# Autodesk Inventor assembly: motor
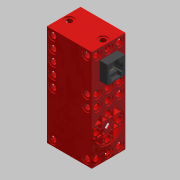
[picture p0: Inventor's stored thumbnail of the model, 180x180]
Saved by Autodesk Inventor 2019.3 (Build 233278000, 278)
## iProperties
Created: 2019-03-27
Part Number: motor
Description: STEP AP214
Document SubType Name: Assembly
Designer: Varga Daniel
Sending System: SolidWorks 2019
Preprocessor: SwSTEP 2.0
Title: motor_.STEP
Revision Number: ANY
## Documents named in this file (10)
- C:\!_Dani\!_cloud\OneDrive\!_munka\Revolution\RevvyDemoKit\Structural parts\Kickstarter videos\Motor\motor.iam
- C:\!_Dani\!_cloud\OneDrive\!_munka\Revolution\RevvyDemoKit\Structural parts\Kickstarter videos\Motor\rj45_vert.ipt
- C:\!_Dani\!_cloud\OneDrive\!_munka\Revolution\RevvyDemoKit\Structural parts\Kickstarter videos\Motor\MOhA.ipt
- C:\!_Dani\!_cloud\OneDrive\!_munka\Revolution\RevvyDemoKit\Structural parts\Kickstarter videos\Motor\MOcA_1.ipt
- C:\!_Dani\!_cloud\OneDrive\!_munka\Revolution\RevvyDemoKit\Structural parts\Kickstarter videos\Motor\MOcA_2.ipt
- C:\!_Dani\!_cloud\OneDrive\!_munka\Revolution\RevvyDemoKit\Structural parts\Kickstarter videos\Motor\ff130-13200.ipt
- C:\!_Dani\!_cloud\OneDrive\!_munka\Revolution\RevvyDemoKit\Structural parts\Kickstarter videos\Motor\Magnet_ring^motor.ipt
- C:\!_Dani\!_cloud\OneDrive\!_munka\Revolution\RevvyDemoKit\Structural parts\Kickstarter videos\Motor\gearbox^motor.ipt
- C:\!_Dani\!_cloud\OneDrive\!_munka\Revolution\RevvyDemoKit\Structural parts\Kickstarter videos\Motor\PCB^motor.ipt
- C:\!_Dani\!_cloud\OneDrive\!_munka\Revolution\RevvyDemoKit\Structural parts\Kickstarter videos\Motor\small_gear.ipt
## Components (10 placed, 10 different names)
1. rj45_vert_1
2. MOhA_2
3. MOhA_3
4. MOcA_1_4
5. MOcA_2_5
6. ff130-13200_6 — Flush:1, Flush:2, Mate:1, Mate:2, Flush:3, Mate:3, Flush:4
7. Magnet_ring^motor_7 — Mate:2, Flush:3
8. gearbox^motor_8 — Flush:1, Flush:2, Mate:1
9. PCB^motor_9
10. small_gear:1 — Mate:3, Flush:4
## Relationships (7: Flush 4, Mate 3)
- Flush:1 (2.3 mm): ff130-13200_6 ↔ gearbox^motor_8
- Flush:2 (-25 mm): ff130-13200_6 ↔ gearbox^motor_8
- Mate:1: ff130-13200_6 ↔ gearbox^motor_8
- Mate:2: ff130-13200_6 ↔ Magnet_ring^motor_7
- Flush:3 (9 mm): ff130-13200_6 ↔ Magnet_ring^motor_7
- Mate:3: ff130-13200_6 ↔ small_gear:1
- Flush:4 (0.5 mm): ff130-13200_6 ↔ small_gear:1
